# Autodesk Inventor assembly: Link_Supporter_6
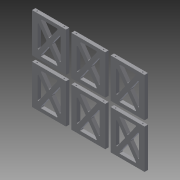
[picture p0: Inventor's stored thumbnail of the model, 180x180]
Saved by Autodesk Inventor 2013 (Build 170138000, 138)
## iProperties
Created: 2014-05-21
Part Number: Link_Supporter_6
Document SubType Name: Assembly
Designer: andou
Author: andou
## Documents named in this file (2)
- C:\Users\andou\Documents\Inventor\RoboticsProject\project_4\Robot\Arm\Link_Supporter_6.iam
- C:\Users\andou\Documents\Inventor\RoboticsProject\project_4\Robot\Arm\Link_Supporter.ipt
## Components (6 placed, 1 different names)
1. Link_Supporter:1
2. Link_Supporter:2
3. Link_Supporter:3
4. Link_Supporter:4
5. Link_Supporter:5
6. Link_Supporter:6
## Component patterns: (6 elements, first: Link_Supporter:1)
